# Autodesk Inventor assembly: Intro a ensamble Sebastian Bermúdez
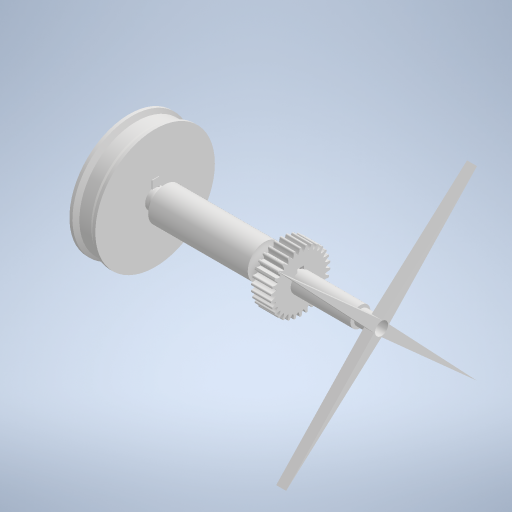
[picture p0: Inventor's stored thumbnail of the model, 512x512]
Saved by Autodesk Inventor 2024.2 (Build 282272000, 272)
## iProperties
Created: 2024-03-31
Part Number: Intro a ensamble Sebastian Bermúdez
Document SubType Name: Assembly
Designer: sberl
Mass: 425.889 g
Surface Area: 649.366 cm^2
Volume: 425.889 cm^3
Density: 1 g/cm^3
Author: sberl
## Documents named in this file (9)
- C:\Users\sberl\Downloads\Intro a ensamble Sebastian Bermúdez.iam
- C:\Users\sberl\Downloads\EJE_CUÑEROS.ipt
- C:\Users\sberl\Downloads\ENGRANE.ipt
- C:\Users\sberl\Downloads\POLEA.ipt
- C:\Users\sberl\Downloads\CUÑA.ipt
- C:\Users\sberl\Downloads\Assembly13.iam
- C:\Users\sberl\Downloads\Assembly14.iam
- C:\Users\sberl\Downloads\apoyo ventilador.ipt
- C:\Users\sberl\Downloads\Ventilador.ipt
## Components (8 placed, 8 different names)
1. EJE_CUÑEROS:1 — Mate:1, Mate:2, Mate:3, Mate:4, Mate:5, Mate:6, Mate:7, Mate:8
2. ENGRANE:1 — Mate:1, Mate:2
3. POLEA:1 — Mate:3, Mate:6
4. CUÑA:1 — Mate:4, Mate:5
5. Assembly13:1 [sub-assembly]
6. Assembly14:1 [sub-assembly]
7. apoyo ventilador:1 — Mate:7, Mate:8, Mate:9, Rotation:1
8. Ventilador:1 — Mate:9, Rotation:1
## Relationships (10: Mate 9, RelateRotation 1)
- Mate:1: EJE_CUÑEROS:1 ↔ ENGRANE:1
- Mate:2: EJE_CUÑEROS:1 ↔ ENGRANE:1
- Mate:3: EJE_CUÑEROS:1 ↔ POLEA:1
- Mate:4: EJE_CUÑEROS:1 ↔ CUÑA:1
- Mate:5: EJE_CUÑEROS:1 ↔ CUÑA:1
- Mate:6: EJE_CUÑEROS:1 ↔ POLEA:1
- Mate:7: EJE_CUÑEROS:1 ↔ apoyo ventilador:1
- Mate:8: EJE_CUÑEROS:1 ↔ apoyo ventilador:1
- Mate:9: apoyo ventilador:1 ↔ Ventilador:1
- Rotation:1 [RelateRotation] (0.65 ul): apoyo ventilador:1 ↔ Ventilador:1
